# Autodesk Inventor assembly: Sideways pulley mount
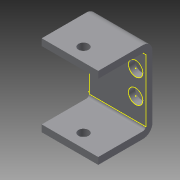
[picture p0: Inventor's stored thumbnail of the model, 180x180]
Saved by Autodesk Inventor 2013 (Build 170138000, 138)
## iProperties
Created: 2013-02-07
Part Number: Sideways pulley mount
Document SubType Name: Assembly
Designer: Arpan
Mass: 9.61328 g
Surface Area: 67.8393 cm^2
Volume: 9.61328 cm^3
Density: 1 g/cm^3
Author: Arpan
## Documents named in this file (4)
- C:\Users\Arpan\Documents\GitHub\frc2013CAD\Cimber actual\Sideways pulley mount.iam
- C:\Users\Arpan\Documents\GitHub\frc2013CAD\Cimber actual\pulley mount. actual sideways ipt.ipt
- C:\Users\Arpan\Documents\GitHub\frc2013CAD\Cimber actual\3 16ths shaft.ipt
- C:\Users\Arpan\Documents\GitHub\frc2013CAD\Cimber actual\1 8th pulley.ipt
## Components (3 placed, 3 different names)
1. pulley mount. actual sideways ipt:1 — Mate:1, Flush:1, Mate:3
2. 3 16ths shaft:1 — Mate:1, Flush:1, Mate:2
3. 1 8th pulley:1 — Mate:2, Mate:3
## Relationships (4: Mate 3, Flush 1)
- Mate:1: pulley mount. actual sideways ipt:1 ↔ 3 16ths shaft:1
- Flush:1: pulley mount. actual sideways ipt:1 ↔ 3 16ths shaft:1
- Mate:2: 3 16ths shaft:1 ↔ 1 8th pulley:1
- Mate:3 (11.2268 mm): pulley mount. actual sideways ipt:1 ↔ 1 8th pulley:1
